# Autodesk Inventor assembly: Build
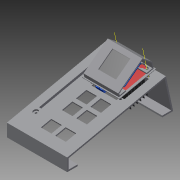
[picture p0: Inventor's stored thumbnail of the model, 180x180]
Saved by Autodesk Inventor 2015 (Build 190159000, 159)
## iProperties
Created: 2022-04-16
Part Number: Build
Document SubType Name: Assembly
Designer: Jan
Author: Jan
## Documents named in this file (6)
- C:\Users\Jan\Ordnerstruktur\CodeRepository\Git\deej\3D_Design\Build.iam
- C:\Users\Jan\Ordnerstruktur\CodeRepository\Git\deej\3D_Design\Main_Corpse.ipt
- C:\Users\Jan\Ordnerstruktur\CodeRepository\Git\deej\3D_Design\Imported Components\L298N Motor Driver\L298N Motor Driver.ipt
- C:\Users\Jan\Ordnerstruktur\CodeRepository\Git\deej\3D_Design\1-3-tft-ips-module-st7789-1.snapshot.7\Imported Components\1.3 TFT IPS - Module\1.3 TFT IPS - Module.iam
- C:\Users\Jan\Ordnerstruktur\CodeRepository\Git\deej\3D_Design\DisplayMount.ipt
- C:\Users\Jan\Ordnerstruktur\CodeRepository\Git\deej\3D_Design\DistancePlate.ipt
## Components (5 placed, 5 different names)
1. Main_Corpse:1 — Mate:16, Mate:17
2. L298N Motor Driver:1 — Mate:14, Mate:15, Mate:18, Mate:19, Mate:20
3. 1.3 TFT IPS - Module:1 [sub-assembly] — Mate:8, Mate:9
4. DisplayMount:1 — Mate:8, Mate:9, Mate:14, Mate:15, Mate:16, Mate:17, Mate:22
5. DistancePlate:1 — Mate:18, Mate:19, Mate:20, Mate:22
## Relationships (10: Mate 10)
- Mate:8: 1.3 TFT IPS - Module:1 ↔ DisplayMount:1
- Mate:9: 1.3 TFT IPS - Module:1 ↔ DisplayMount:1
- Mate:14: L298N Motor Driver:1 ↔ DisplayMount:1
- Mate:15: L298N Motor Driver:1 ↔ DisplayMount:1
- Mate:16: Main_Corpse:1 ↔ DisplayMount:1
- Mate:17: Main_Corpse:1 ↔ DisplayMount:1
- Mate:18: L298N Motor Driver:1 ↔ DistancePlate:1
- Mate:19: L298N Motor Driver:1 ↔ DistancePlate:1
- Mate:20: L298N Motor Driver:1 ↔ DistancePlate:1
- Mate:22: DisplayMount:1 ↔ DistancePlate:1
